# Autodesk Inventor assembly: ASY SLM 1110 MAIN FRAME
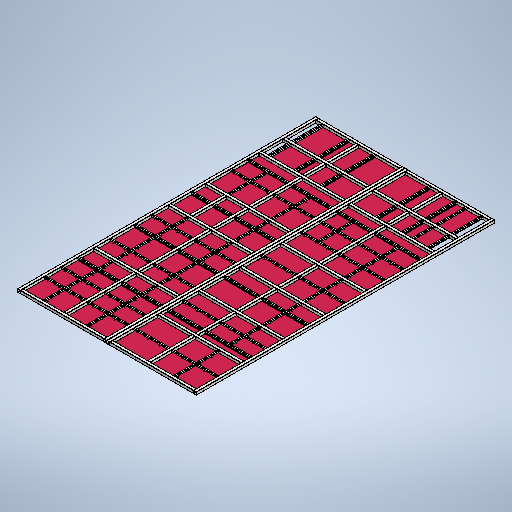
[picture p0: Inventor's stored thumbnail of the model, 512x512]
Saved by Autodesk Inventor 2025.3 (Build 293356030, 356C)
## iProperties
Created: 2025-12-15
Part Number: ASY SLM 1110 MAIN FRAME
Document SubType Name: Assembly
Designer: admin
Mass: 1.03915e+06 g
Surface Area: 883173 cm^2
Volume: 132376 cm^3
Density: 7.85 g/cm^3
_SolveAssemblyDoc: Frame Generator Solve Assembly
_Version: 25.0.0
Author: admin
## Documents named in this file (13)
- C:\Users\admin\Documents\Inventor\SLM-Salemal\ASY SLM 1110 MAIN FRAME.iam
- C:\Users\admin\Documents\Inventor\SLM-Salemal\Frame\PNS-1100 FRAME Main sketch.ipt
- C:\Users\admin\Documents\Inventor\SLM-Salemal\ASY SLM 1110 MAIN FRAME\Frame\Frame 1768306688236.iam
- C:\Users\admin\Documents\Inventor\SLM-Salemal\SLM-frame 1.1 floor sheet 4.ipt
- C:\Users\admin\Documents\Inventor\SLM-Salemal\SLM-frame 1.1 floor sheet 5.ipt
- C:\Users\admin\Documents\Inventor\SLM-Salemal\SLM-frame 1.1 floor sheet 4_CPY.ipt
- C:\Users\admin\Documents\Inventor\SLM-Salemal\SLM-frame 1.1 floor sheet 2.ipt
- C:\Users\admin\Documents\Inventor\SLM-Salemal\SLM-frame 1.1 floor sheet 3.ipt
- C:\Users\admin\Documents\Inventor\SLM-Salemal\SLM-frame 1.1 floor sheet.ipt
- C:\Users\admin\Documents\Inventor\SLM-Salemal\SLM-frame 2 floor sheet 6.ipt
- C:\Users\admin\Documents\Inventor\SLM-Salemal\SLM-frame 2 floor sheet 8.ipt
- C:\Users\admin\Documents\Inventor\SLM-Salemal\SLM-frame 2 floor sheet 9.ipt
- C:\Users\admin\Documents\Inventor\SLM-Salemal\SLM-frame 2 floor sheet 10.ipt
## Components (18 placed, 12 different names)
1. PNS-1100 FRAME Main sketch:1
2. Frame 1768306688236:1 [sub-assembly] — Mate:2, Mate:3, Mate:4, Mate:5, Mate:6, Mate:7
3. GnG L.1 floor sheet:1 — Mate:2, Mate:3, Rigid:3, Mate:7
4. GnG L.2 floor sheet:1 — Rigid:3, Rigid:4
5. GnG L.3 floor sheet:1 — Rigid:4, Rigid:5
6. GnG L.4 floor sheet:1 — Rigid:1, Rigid:5
7. GnG L.5:1 — Rigid:1, Rigid:9, Rigid:18
8. SLM-frame 1.1 floor sheet 4_CPY:1 — Mate:4, Mate:5, Mate:6, Rigid:16
9. GnG frame 2 floor sheet 8:1 — Rigid:16, Rigid:19
10. GnG frame 2 floor sheet 9:1 — Rigid:19, Rigid:20
11. GnG frame 2 floor sheet 6:1 — Rigid:20
12. GnG L.5:2 — Rigid:18
13. GnG X.6 floor sheet:1 — Rigid:7
14. GnG X.6 floor sheet:2 — Rigid:6, Rigid:7
15. GnG X.6 floor sheet:3 — Rigid:6, Rigid:9, Rigid:17
16. GnG X.6 floor sheet:4 — Rigid:14, Rigid:17
17. GnG X.6 floor sheet:5 — Rigid:14, Rigid:15
18. GnG X.6 floor sheet:6 — Rigid:15
## Relationships (20: WeldJoint 14, Mate 6)
- Rigid:1 [WeldJoint] (20 mm): GnG L.4 floor sheet:1 ↔ GnG L.5:1
- Mate:2 (-30 mm): Frame 1768306688236:1 ↔ GnG L.1 floor sheet:1
- Mate:3 (-30 mm): Frame 1768306688236:1 ↔ GnG L.1 floor sheet:1
- Rigid:3 [WeldJoint] (20 mm): GnG L.1 floor sheet:1 ↔ GnG L.2 floor sheet:1
- Rigid:4 [WeldJoint] (20 mm): GnG L.2 floor sheet:1 ↔ GnG L.3 floor sheet:1
- Rigid:5 [WeldJoint] (20 mm): GnG L.3 floor sheet:1 ↔ GnG L.4 floor sheet:1
- Rigid:6 [WeldJoint] (20 mm): GnG X.6 floor sheet:2 ↔ GnG X.6 floor sheet:3
- Rigid:7 [WeldJoint] (20 mm): GnG X.6 floor sheet:1 ↔ GnG X.6 floor sheet:2
- Rigid:9 [WeldJoint] (20 mm): GnG L.5:1 ↔ GnG X.6 floor sheet:3
- Rigid:14 [WeldJoint] (20 mm): GnG X.6 floor sheet:4 ↔ GnG X.6 floor sheet:5
- Rigid:15 [WeldJoint] (20 mm): GnG X.6 floor sheet:5 ↔ GnG X.6 floor sheet:6
- Mate:4: Frame 1768306688236:1 ↔ SLM-frame 1.1 floor sheet 4_CPY:1
- Mate:5 (-30 mm): Frame 1768306688236:1 ↔ SLM-frame 1.1 floor sheet 4_CPY:1
- Mate:6 (-30 mm): Frame 1768306688236:1 ↔ SLM-frame 1.1 floor sheet 4_CPY:1
- Rigid:16 [WeldJoint] (20 mm): SLM-frame 1.1 floor sheet 4_CPY:1 ↔ GnG frame 2 floor sheet 8:1
- Rigid:17 [WeldJoint] (100 mm): GnG X.6 floor sheet:3 ↔ GnG X.6 floor sheet:4
- Rigid:18 [WeldJoint] (100 mm): GnG L.5:1 ↔ GnG L.5:2
- Rigid:19 [WeldJoint] (20 mm): GnG frame 2 floor sheet 8:1 ↔ GnG frame 2 floor sheet 9:1
- Rigid:20 [WeldJoint] (20 mm): GnG frame 2 floor sheet 9:1 ↔ GnG frame 2 floor sheet 6:1
- Mate:7: Frame 1768306688236:1 ↔ GnG L.1 floor sheet:1
